# Autodesk Inventor assembly: Trochoidal_Roller_Pinion_Rack
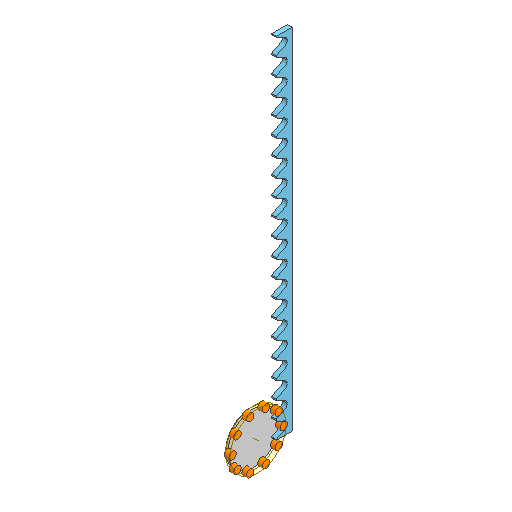
[picture p0: Inventor's stored thumbnail of the model, 512x512]
Saved by Autodesk Inventor 2025.3 (Build 293356000, 356)
## iProperties
Created: 2026-06-13
Part Number: Trochoidal_Roller_Pinion_Rack
Document SubType Name: Assembly
Designer: PC
Author: PC
## Documents named in this file (3)
- C:\Users\PC\Data\Documents\git\Trochoidal_Roller_Pinion_Rack_Design\Trochoidal_Roller_Pinion_Rack.iam
- C:\Users\PC\Data\Documents\git\Trochoidal_Roller_Pinion_Rack_Design\Roller Pinion.ipt
- C:\Users\PC\Data\Documents\git\Trochoidal_Roller_Pinion_Rack_Design\Rack.ipt
## Components (2 placed, 2 different names)
1. Roller Pinion:1 — Flush:1, Mate:3, Angle:1, Rotation/Translation:1, Mate:6, Mate:7
2. Rack:1 — Flush:2, Flush:3, Flush:5, Rotation/Translation:1
## Relationships (10: Flush 5, Mate 3, Angle 1, RelateRotateTranslate 1)
- Flush:1: Roller Pinion:1
- Flush:2: Rack:1
- Flush:3: Rack:1
- Flush:4 (60 mm)
- Mate:3: Roller Pinion:1
- Angle:1 (0 deg): Roller Pinion:1
- Flush:5: Rack:1
- Rotation/Translation:1 [RelateRotateTranslate] (376.9911 mm): Roller Pinion:1 ↔ Rack:1
- Mate:6: Roller Pinion:1
- Mate:7: Roller Pinion:1
## Named parameters: R = 60 mm, z = 10, module = 11 mm, Simulation_Timeline = 0
